# Autodesk Inventor assembly: RA15 Kinematic Model
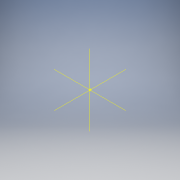
[picture p0: Inventor's stored thumbnail of the model, 180x180]
Saved by Autodesk Inventor 2019 (Build 230136000, 136)
## iProperties
Created: 2020-08-30
Part Number: RA15 Kinematic Model
Document SubType Name: Assembly
Designer: Daniel
d_1: 176.000 mm
r_1: 0.000 mm
alpha_1: 90.00 deg
theta_1: 0.00 deg
d_2: 0.000 mm
r_2: 208.000 mm
alpha_2: 0.00 deg
theta_2: 90.00 deg
d_3: 0.000 mm
r_3: 48.000 mm
alpha_3: 90.00 deg
theta_3: 0.00 deg
d_4: 184.000 mm
r_4: 0.000 mm
alpha_4: 90.00 deg
theta_4: 0.00 deg
d_5: 0.000 mm
r_5: 0.000 mm
alpha_5: -90.00 deg
theta_5: 0.00 deg
d_6: 112.000 mm
r_6: 0.000 mm
alpha_6: 0.00 deg
theta_6: 0.00 deg
Author: Daniel
## Documents named in this file (2)
- B:\Projects\Robotics\Mindstorms\RA15\kinematic model\RA15 Kinematic Model.iam
- B:\Projects\Robotics\Mindstorms\RA15\kinematic model\dh_params.xlsx
## Named parameters: d_1 = 176 mm, r_1 = 0 mm, alpha_1 = 90 deg, theta_1 = 0 deg, d_2 = 0 mm, r_2 = 208 mm, alpha_2 = 0 deg, theta_2 = 90 deg, d_3 = 0 mm, r_3 = 48 mm, alpha_3 = 90 deg, theta_3 = 0 deg, d_4 = 184 mm, r_4 = 0 mm, alpha_4 = 90 deg, theta_4 = 0 deg, d_5 = 0 mm, r_5 = 0 mm, alpha_5 = -90 deg, theta_5 = 0 deg, d_6 = 112 mm, r_6 = 0 mm, alpha_6 = 0 deg, theta_6 = 0 deg
